# Autodesk Inventor assembly: Battery
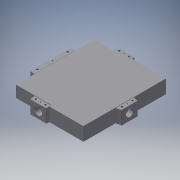
[picture p0: Inventor's stored thumbnail of the model, 180x180]
Saved by Autodesk Inventor 2016 (Build 200138000, 138)
## iProperties
Created: 2015-09-14
Part Number: Battery
Document SubType Name: Assembly
Designer: lachesis
Author: lachesis
## Documents named in this file (4)
- C:\Users\lachesis\git\Swarmie-Build\Swarmie-Assembly\Assemblies\Battery.iam
- C:\Users\lachesis\git\Swarmie-Build\Swarmie-Assembly\Parts\BatteryBase.ipt
- C:\Users\lachesis\git\Swarmie-Build\Swarmie-Assembly\Parts\BatteryInBag.ipt
- C:\Users\lachesis\git\Swarmie-Build\Swarmie-Assembly\Parts\BatteryBrace.ipt
## Components (3 placed, 3 different names)
1. BatteryBase:1 — Mate:1, Mate:2, Mate:3
2. BatteryInBag:1 — Mate:1, Mate:2, Mate:3, Rigid:1
3. BatteryBrace:1 — Rigid:1
## Relationships (4: Mate 3, WeldJoint 1)
- Mate:1: BatteryBase:1 ↔ BatteryInBag:1
- Mate:2: BatteryBase:1 ↔ BatteryInBag:1
- Mate:3: BatteryBase:1 ↔ BatteryInBag:1
- Rigid:1 [WeldJoint]: BatteryInBag:1 ↔ BatteryBrace:1
